# Autodesk Inventor assembly: Chalk Applicator
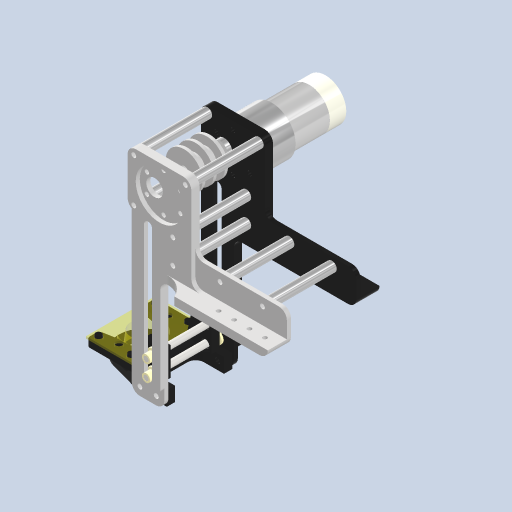
[picture p0: Inventor's stored thumbnail of the model, 512x512]
Saved by Autodesk Inventor 2024 (Build 280153000, 153)
## iProperties
Created: 2023-12-18
Part Number: Chalk Applicator
Document SubType Name: Assembly
Designer: greg
Author: greg
## Documents named in this file (10)
- C:\Users\Greg\Documents\Inventor\Capstone\Chalk Applicator\Chalk Applicator.iam
- C:\Users\Greg\Documents\Inventor\Capstone\Chalk Applicator\Cross Shaft.iam
- C:\Users\Greg\Documents\Inventor\Capstone\Chalk Applicator\Standoff.ipt
- C:\Users\Greg\Documents\Inventor\Capstone\Chalk Applicator\Carriage.ipt
- C:\Users\Greg\Documents\Inventor\Capstone\Chalk Applicator\Gripper.ipt
- C:\Users\Greg\Documents\Inventor\Capstone\Chalk Applicator\Lower Guide.ipt
- C:\Users\Greg\Documents\Inventor\Capstone\Chalk Applicator\Side Plate 2.0.ipt
- C:\Users\Greg\Documents\Inventor\Capstone\Chalk Applicator\Vince-Motor.ipt
- C:\Users\Greg\Documents\Inventor\Capstone\Chalk Applicator\Side Plate 2.0_MIR.ipt
- C:\Users\Greg\Documents\Inventor\Capstone\Chalk Applicator\PulleyV2.ipt
## Components (16 placed, 9 different names)
1. Cross Shaft:1 [sub-assembly] — Mate:29, Tangent:2, Mate:31
2. Cross Shaft:2 [sub-assembly] — Mate:28, Mate:30, Tangent:1, Mate:32
3. Standoff:4 — Insert:19, Insert:20
4. Carriage:1 — Mate:28, Mate:29, Mate:30, Insert:11, Insert:12
5. Gripper:1 — Insert:11, Insert:12
6. Lower Guide:1 — Insert:13, Insert:14, Insert:17, Insert:18
7. Side Plate 2.0:1 — Insert:13, Insert:14, Tangent:1, Tangent:2, Mate:31, Mate:32, Insert:15, Insert:16, Insert:19, Insert:21, Insert:22, Insert:23, Insert:24, Insert:25, Insert:26
8. Vince-Motor:1 — Insert:15, Insert:16, Mate:33
9. Side Plate 2.0_MIR:1 — Insert:17, Insert:18, Insert:20
10. PulleyV2:1 — Mate:33
11. Standoff:5 — Insert:22
12. Standoff:6 — Insert:21
13. Standoff:7 — Insert:23
14. Standoff:8 — Insert:26
15. Standoff:9 — Insert:25
16. Standoff:10 — Insert:24
## Relationships (24: Insert 16, Mate 6, Tangent 2)
- Mate:28: Cross Shaft:2 ↔ Carriage:1
- Mate:29: Cross Shaft:1 ↔ Carriage:1
- Mate:30 (1.5875 mm): Cross Shaft:2 ↔ Carriage:1
- Insert:11: Carriage:1 ↔ Gripper:1
- Insert:12: Carriage:1 ↔ Gripper:1
- Insert:13: Lower Guide:1 ↔ Side Plate 2.0:1
- Insert:14: Lower Guide:1 ↔ Side Plate 2.0:1
- Tangent:1: Cross Shaft:2 ↔ Side Plate 2.0:1
- Tangent:2: Cross Shaft:1 ↔ Side Plate 2.0:1
- Mate:31: Cross Shaft:1 ↔ Side Plate 2.0:1
- Mate:32: Cross Shaft:2 ↔ Side Plate 2.0:1
- Insert:15: Side Plate 2.0:1 ↔ Vince-Motor:1
- Insert:16: Side Plate 2.0:1 ↔ Vince-Motor:1
- Insert:17: Lower Guide:1 ↔ Side Plate 2.0_MIR:1
- Insert:18: Lower Guide:1 ↔ Side Plate 2.0_MIR:1
- Insert:19: Standoff:4 ↔ Side Plate 2.0:1
- Insert:20: Standoff:4 ↔ Side Plate 2.0_MIR:1
- Insert:21: Side Plate 2.0:1 ↔ Standoff:6
- Insert:22: Side Plate 2.0:1 ↔ Standoff:5
- Insert:23: Side Plate 2.0:1 ↔ Standoff:7
- Insert:24: Side Plate 2.0:1 ↔ Standoff:10
- Insert:25: Side Plate 2.0:1 ↔ Standoff:9
- Insert:26: Side Plate 2.0:1 ↔ Standoff:8
- Mate:33: Vince-Motor:1 ↔ PulleyV2:1
